# Autodesk Inventor assembly: TruckAssembly
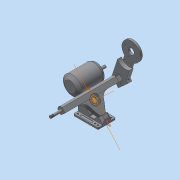
[picture p0: Inventor's stored thumbnail of the model, 180x180]
Saved by Autodesk Inventor 2017 (Build 210142000, 142)
## iProperties
Created: 2015-12-02
Part Number: TruckAssembly
Document SubType Name: Assembly
Designer: JoshuaYuan
Author: JoshuaYuan
## Documents named in this file (7)
- C:\Other Project Stuff\Longboard\TruckAssembly.iam
- C:\Other Project Stuff\Longboard\50cal_truck.ipt
- C:\Other Project Stuff\Longboard\50cal_baseplate.ipt
- C:\Other Project Stuff\Longboard\MotorMountAssembly.iam
- C:\Other Project Stuff\Longboard\motor.ipt
- C:\Other Project Stuff\Longboard\Wheels.ipt
- C:\Other Project Stuff\Longboard\bearing_ABEC_7.ipt
## Components (7 placed, 7 different names)
1. 50cal_truck:1 — Mate:1, Mate:2, truck axle insert, Flush:1, Mate:3, Mate:4
2. 50cal_baseplate:1 — Mate:1, Mate:2
3. MotorMountAssembly:1 [sub-assembly] — Insert:5, Flush:1, Mate:3, Mate:4
4. Wheels:1 — outer bearing insert, inner bearing insert, truck axle insert
5. outer bearing — outer bearing insert
6. inner bearing — inner bearing insert
7. motor:1 — Insert:5
## Relationships (9: Mate 4, Insert 4, Flush 1)
- Mate:1: 50cal_truck:1 ↔ 50cal_baseplate:1
- Mate:2: 50cal_truck:1 ↔ 50cal_baseplate:1
- outer bearing insert [Insert]: Wheels:1 ↔ outer bearing
- inner bearing insert [Insert]: Wheels:1 ↔ inner bearing
- truck axle insert [Insert] (2 mm): 50cal_truck:1 ↔ Wheels:1
- Insert:5: MotorMountAssembly:1 ↔ motor:1
- Flush:1: 50cal_truck:1 ↔ MotorMountAssembly:1
- Mate:3: 50cal_truck:1 ↔ MotorMountAssembly:1
- Mate:4: 50cal_truck:1 ↔ MotorMountAssembly:1
